# Autodesk Inventor assembly: SSE2BSLZ8-140
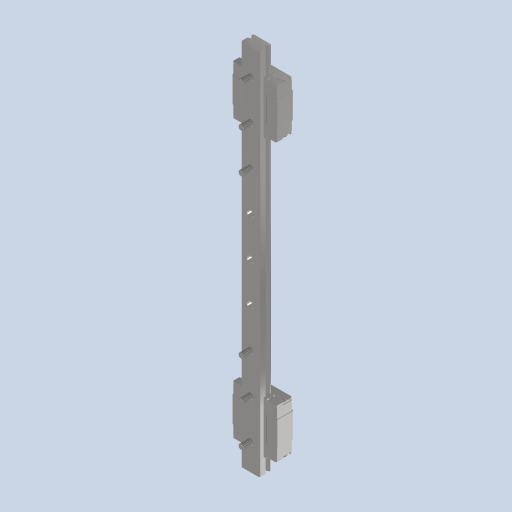
[picture p0: Inventor's stored thumbnail of the model, 512x512]
Saved by Autodesk Inventor 2023 (Build 270158000, 158)
## iProperties
Category: PARTsolutions
Company: MISUMI
Created: 2024-12-13
Part Number: SSE2BSLZ8-140
Catalog Web Link: www.cadenas.de
Description: SSEBSLZ, SSEBSLZ-MX, SSE2BSLZ, SSE2BSLZ-MX-Miniature Linear Guides - Short Blocks - Light Preload/Slight Clearance - Standard Grade - Configurable
Vendor: MISUMI
Document SubType Name: Assembly
Designer: psAdmin
Manufacturer: MISUMI
Mass: 58.3972 g
Surface Area: 73.7645 cm^2
Volume: 7.29965 cm^3
Density: 8 g/cm^3
PSOL_IDENT_0: {$CADENAS_DATA/23d-libs/misumi/metric/06_linear_guides/sebslz_asmtab.prj},252 {VTYP=3D},{STYP=ASSTAB
PSOL_IDENT_1: },{NB=SSE2BSLZ8-140},{LINA=SSE2BSLZ8-140},{NN=SSEBSLZ, SSEBSLZ-MX, SSE2BSLZ, SSE2BSLZ-MX},{DATE=04.0
PSOL_IDENT_2: 4.2024 07:13:14},{GEOMDATE=06.03.2024 06:19:47},{VERSION=},{LINEID=90},{WBVAR=TS,ST,MAT,MX,NOB,GREAS
PSOL_IDENT_3: E,L,ALT1,ALT4},{WBNUMERIC=L}  {NB=SSE2BSLZ8-140},{LINA=SSE2BSLZ8-140},{KT=DUMMY},{PN=SSE2BSLZ8-140},
PSOL_IDENT_4: {RT=B},{TS=Z},{TS1= 'Z','Standard' },{ST=S},{ST1='S', 'w/o Surface Treatment'},{TYPE=SSE2BSLZ},{MAT=
PSOL_IDENT_5: S},{MX=},{MXALG= '','w/o MX(Lubrication unit)' },{NOB=2},{H=8},{GREASE=},{GREASEALG='','Normal', 'L'
PSOL_IDENT_6: , 'L Type Greased ', 'G', 'G Type Greased', 'Y', 'Y Type Greased', 'H', 'H Type Greased'},{LT=Confi
PSOL_IDENT_7: gurable},{L=140},{HARD=56HRC~},{W=17},{L1=19.6},{B=12},{C=8},{SLL=M2x2.5},{L2=9.6},{K=6.5},{CBB=0.3}
PSOL_IDENT_8: ,{W1=7},{W2=5.0},{H1=4.7},{CAA=0.3},{DD1DD2HH=2.4x4.2x2.3},{F=15},{G=10},{ALT1=},{ALT1ALG= '', 'w/o
PSOL_IDENT_9: MC (Tapped Holes)' },{MC=M3},{MC1=3.0},{M=9},{LL=L},{L0=[56:69/1],[71:84/1],[86:99/1],[101:114/1],[1
PSOL_IDENT_10: 16:129/1],[131:144/1],[146:159/1],[161:174/1],[176:189/1],[191:204/1],[206:219/1],[221:234/1],[236:2
PSOL_IDENT_11: 49/1],[251:264/1],[266:279/1],[281:294/1],[296:309/1]},{REC1=   '','N/A'    },{ALT4=},{ALT4ALG= '','
PSOL_IDENT_12: N/A' },{PPATH=sebslz_series/sebslz_asmtpl.prj}
NB: SSE2BSLZ8-140
NN: SSEBSLZ, SSEBSLZ-MX, SSE2BSLZ, SSE2BSLZ-MX
NT: Miniature Linear Guides - Short Blocks - Light Preload/Slight Clearance - Standard Grade - Configurable
NBSYN: $PN.
LINA: SSE2BSLZ8-140
CATALOG: Misumi
PN: SSE2BSLZ8-140
MAT: Stainless Steel
MX: w/o MX(Lubrication unit)
NOB: 2
H: 8
GREASE: Normal
L: 140
W: 17
L1: 19.6
B: 12
C: 8
SLL: M2x2.5
L2: 9.6
K: 6.5
CBB: 0.3
W1: 7
W2: 5
H1: 4.7
CAA: 0.3
DD1DD2HH: 2.4x4.2x2.3
F: 15
G: 10
ALT1: w/o MC (Tapped Holes)
ALT4: N/A
SUPPLIER: MISUMI
ARTICLENO: SSE2BSLZ8-140
BOMINFO: SSE2BSLZ8-140
CREATOR: CADENAS GmbH
Title: SSE2BSLZ8-140
Author: Cadenas PARTsolutions
Comments: Miniature Linear Guides - Short Blocks - Light Preload/Slight Clearance - Standard Grade - Configurable
## Documents named in this file (4)
- D:\GitHub\inventor\syu-si\OfficeRobot\ReadyMade\linear_guide\SSE2BSLZ8-140\SSE2BSLZ8-140.iam
- D:\GitHub\inventor\syu-si\OfficeRobot\ReadyMade\linear_guide\SSE2BSLZ8-140\SSE2BLZ8-140_r1.ipt
- D:\GitHub\inventor\syu-si\OfficeRobot\ReadyMade\linear_guide\SSE2BSLZ8-140\SEBSZ8_b.ipt
- D:\GitHub\inventor\syu-si\OfficeRobot\ReadyMade\linear_guide\SSE2BSLZ8-140\BOLT2-6.ipt
## Components (9 placed, 3 different names)
1. SSE2BLZ8-140_r1:1 — to_block_Z@1 <-> to_rail_Z@2, to_block_YZ@1 <-> to_rail_YZ@2, to_block_2_Z@1 <-> to_rail_Z@3, to_block_2_YZ@1 <-> to_rail_YZ@3, to_bolt_1_Z@1 <-> to_cp_Z@4, to_bolt_1_YZ@1 <-> to_cp_YZ@4, to_bolt_2_Z@1 <-> to_cp_Z@5, to_bolt_2_YZ@1 <-> to_cp_YZ@5, to_bolt_3_Z@1 <-> to_cp_Z@6, to_bolt_3_YZ@1 <-> to_cp_YZ@6, to_bolt_7_Z@1 <-> to_cp_Z@10, to_bolt_7_YZ@1 <-> to_cp_YZ@10, to_bolt_8_Z@1 <-> to_cp_Z@11, to_bolt_8_YZ@1 <-> to_cp_YZ@11, to_bolt_9_Z@1 <-> to_cp_Z@12, to_bolt_9_YZ@1 <-> to_cp_YZ@12
2. SEBSZ8_b:1 — to_block_Z@1 <-> to_rail_Z@2, to_block_YZ@1 <-> to_rail_YZ@2
3. SEBSZ8_b:2 — to_block_2_Z@1 <-> to_rail_Z@3, to_block_2_YZ@1 <-> to_rail_YZ@3
4. BOLT2-6:1 — to_bolt_1_Z@1 <-> to_cp_Z@4, to_bolt_1_YZ@1 <-> to_cp_YZ@4
5. BOLT2-6:2 — to_bolt_2_Z@1 <-> to_cp_Z@5, to_bolt_2_YZ@1 <-> to_cp_YZ@5
6. BOLT2-6:3 — to_bolt_3_Z@1 <-> to_cp_Z@6, to_bolt_3_YZ@1 <-> to_cp_YZ@6
7. BOLT2-6:7 — to_bolt_7_Z@1 <-> to_cp_Z@10, to_bolt_7_YZ@1 <-> to_cp_YZ@10
8. BOLT2-6:8 — to_bolt_8_Z@1 <-> to_cp_Z@11, to_bolt_8_YZ@1 <-> to_cp_YZ@11
9. BOLT2-6:9 — to_bolt_9_Z@1 <-> to_cp_Z@12, to_bolt_9_YZ@1 <-> to_cp_YZ@12
## Relationships (16: Mate 8, Angle 8)
- to_block_Z@1 <-> to_rail_Z@2 [Mate]: SSE2BLZ8-140_r1:1 ↔ SEBSZ8_b:1
- to_block_YZ@1 <-> to_rail_YZ@2 [Angle] (180 deg): SSE2BLZ8-140_r1:1 ↔ SEBSZ8_b:1
- to_block_2_Z@1 <-> to_rail_Z@3 [Mate]: SSE2BLZ8-140_r1:1 ↔ SEBSZ8_b:2
- to_block_2_YZ@1 <-> to_rail_YZ@3 [Angle] (180 deg): SSE2BLZ8-140_r1:1 ↔ SEBSZ8_b:2
- to_bolt_1_Z@1 <-> to_cp_Z@4 [Mate]: SSE2BLZ8-140_r1:1 ↔ BOLT2-6:1
- to_bolt_1_YZ@1 <-> to_cp_YZ@4 [Angle] (0 deg): SSE2BLZ8-140_r1:1 ↔ BOLT2-6:1
- to_bolt_2_Z@1 <-> to_cp_Z@5 [Mate]: SSE2BLZ8-140_r1:1 ↔ BOLT2-6:2
- to_bolt_2_YZ@1 <-> to_cp_YZ@5 [Angle] (0 deg): SSE2BLZ8-140_r1:1 ↔ BOLT2-6:2
- to_bolt_3_Z@1 <-> to_cp_Z@6 [Mate]: SSE2BLZ8-140_r1:1 ↔ BOLT2-6:3
- to_bolt_3_YZ@1 <-> to_cp_YZ@6 [Angle] (0 deg): SSE2BLZ8-140_r1:1 ↔ BOLT2-6:3
- to_bolt_7_Z@1 <-> to_cp_Z@10 [Mate]: SSE2BLZ8-140_r1:1 ↔ BOLT2-6:7
- to_bolt_7_YZ@1 <-> to_cp_YZ@10 [Angle] (0 deg): SSE2BLZ8-140_r1:1 ↔ BOLT2-6:7
- to_bolt_8_Z@1 <-> to_cp_Z@11 [Mate]: SSE2BLZ8-140_r1:1 ↔ BOLT2-6:8
- to_bolt_8_YZ@1 <-> to_cp_YZ@11 [Angle] (0 deg): SSE2BLZ8-140_r1:1 ↔ BOLT2-6:8
- to_bolt_9_Z@1 <-> to_cp_Z@12 [Mate]: SSE2BLZ8-140_r1:1 ↔ BOLT2-6:9
- to_bolt_9_YZ@1 <-> to_cp_YZ@12 [Angle] (0 deg): SSE2BLZ8-140_r1:1 ↔ BOLT2-6:9
